# Autodesk Inventor assembly: MotorVezerloHhid
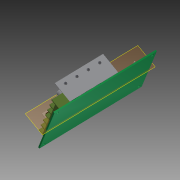
[picture p0: Inventor's stored thumbnail of the model, 180x180]
Saved by Autodesk Inventor 2015 (Build 190159000, 159)
## iProperties
Created: 2014-10-30
Part Number: MotorVezerloHhid
Document SubType Name: Assembly
Designer: laca
Author: laca
## Documents named in this file (3)
- C:\Users\laca\Documents\inventor\iRoobo2014Ver3\MotorVezerloHhid.iam
- C:\Users\laca\Documents\inventor\iRoobo2014Ver3\SzigeteloAlatetTranzisztor.ipt
- C:\Users\laca\Documents\inventor\iRoobo2014Ver3\NyakMotorVezerlo.ipt
## Components (9 placed, 2 different names)
1. NyakMotorVezerlo:1 — Rigid:1, Rigid:2
2. SzigeteloAlatetTranzisztor:5 — Rigid:2
3. SzigeteloAlatetTranzisztor:1 — Rigid:1
4. SzigeteloAlatetTranzisztor:6
5. SzigeteloAlatetTranzisztor:7
6. SzigeteloAlatetTranzisztor:8
7. SzigeteloAlatetTranzisztor:9
8. SzigeteloAlatetTranzisztor:10
9. SzigeteloAlatetTranzisztor:11
## Component patterns: (4 elements, first: SzigeteloAlatetTranzisztor:5 + SzigeteloAlatetTranzisztor:1)
## Relationships (2: WeldJoint 2)
- Rigid:1 [WeldJoint]: NyakMotorVezerlo:1 ↔ SzigeteloAlatetTranzisztor:1
- Rigid:2 [WeldJoint]: NyakMotorVezerlo:1 ↔ SzigeteloAlatetTranzisztor:5
